# Autodesk Inventor assembly: rail_mirrored
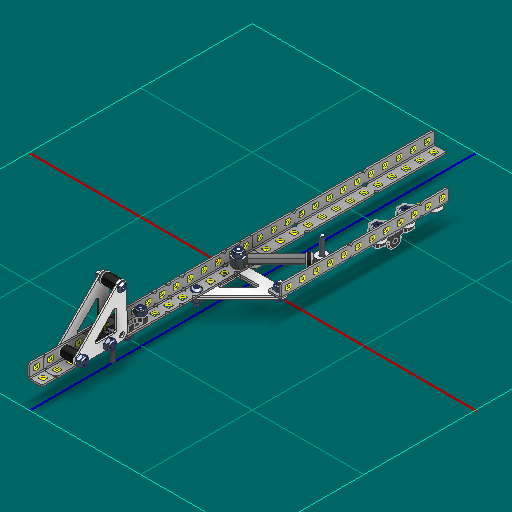
[picture p0: Inventor's stored thumbnail of the model, 512x512]
Saved by Autodesk Inventor 2025 (Build 290162000, 162)
## iProperties
Created: 2024-08-18
Part Number: rail_mirrored
Document SubType Name: Assembly
Designer: averey
Author: averey
## Documents named in this file (21)
- C:\Users\avere\vex_robotics_high_stakes\hardware\cad\ATLAS\chassis\structure\rail_mirrored\rail_mirrored.iam
- C:\Users\avere\vex_robotics_high_stakes\hardware\cad\ATLAS\chassis\structure\rail_mirrored\right_angle_gusset_mirrored.ipt
- C:\Users\avere\vex_robotics_high_stakes\hardware\cad\VEX-CAD-Inventor\Structure\Hardware\Screw Shoulder Robosource\SScrew Shoulder Smooth .500 x .18.ipt
- C:\Users\avere\vex_robotics_high_stakes\hardware\cad\VEX-CAD-Inventor\Structure\Hardware\Screw Shoulder Robosource.ipt
- C:\Users\avere\vex_robotics_high_stakes\hardware\cad\ATLAS\chassis\structure\rail_mirrored\Nut Thin Nylock_mirrored.ipt
- C:\Users\avere\vex_robotics_high_stakes\hardware\cad\ATLAS\chassis\structure\rail_mirrored\Bearing Flat Low Profile_mirrored.ipt
- C:\Users\avere\vex_robotics_high_stakes\hardware\cad\VEX-CAD-Inventor\Structure\Hardware\Screw Steel - Star\SScrew Star Smooth 1.000.ipt
- C:\Users\avere\vex_robotics_high_stakes\hardware\cad\VEX-CAD-Inventor\Structure\Hardware\Screw Steel - Star.ipt
- C:\Users\avere\vex_robotics_high_stakes\hardware\cad\VEX-CAD-Inventor\Structure\Hardware\Screw Shoulder Robosource\SScrew Shoulder Smooth .500 x .04.ipt
- C:\Users\avere\vex_robotics_high_stakes\hardware\cad\ATLAS\chassis\structure\rail_mirrored\Alu Angle 1x1x28_mirrored.ipt
- C:\Users\avere\vex_robotics_high_stakes\hardware\cad\ATLAS\chassis\structure\rail_mirrored\Alu Angle 1x1x15_mirrored.ipt
- C:\Users\avere\vex_robotics_high_stakes\hardware\cad\VEX-CAD-Inventor\Motion\Spacers\Spacer Nylon .500 OD\NSpacer White .500 OD x .125.ipt
- C:\Users\avere\vex_robotics_high_stakes\hardware\cad\VEX-CAD-Inventor\Motion\Spacers\Spacer Nylon .500 OD.ipt
- C:\Users\avere\vex_robotics_high_stakes\hardware\cad\VEX-CAD-Inventor\Structure\Hardware\Screw Steel - Star\SScrew Star Smooth .750.ipt
- C:\Users\avere\vex_robotics_high_stakes\hardware\cad\VEX-CAD-Inventor\Structure\Angle\Aluminum 1x1\Alu Angle 1x1x16.ipt
- C:\Users\avere\vex_robotics_high_stakes\hardware\cad\VEX-CAD-Inventor\Structure\Angle\Aluminum 1x1\Alu Angle 1x1x12.ipt
- C:\Users\avere\vex_robotics_high_stakes\hardware\cad\ATLAS\chassis\structure\standoff_brace_triangle.iam
- C:\Users\avere\vex_robotics_high_stakes\hardware\cad\VEX-CAD-Inventor\Motion\Shaft LS\LS Pillow Bearing Block.ipt
- C:\Users\avere\vex_robotics_high_stakes\hardware\cad\_quick_assemblies\hex_nut_retainer_w_lock_nut.iam
- C:\Users\avere\vex_robotics_high_stakes\hardware\cad\ATLAS\tower\structure\triangle_brace_mirrored.iam
- C:\Users\avere\vex_robotics_high_stakes\hardware\cad\VEX-CAD-Inventor\Structure\Hardware\Nut Thin Nylock.ipt
## Components (29 placed, 17 different names)
1. right_angle_gusset_mirrored:1 — Mate:3, Mate:5, Insert:19, Insert:20
2. right_angle_gusset_mirrored:2 — Mate:3, Mate:5, Insert:11, Insert:12, Insert:23
3. SScrew Shoulder Smooth .500 x .18:1 — Insert:20
4. SScrew Shoulder Smooth .500 x .18:2 — Insert:11, Insert:2, Insert:7
5. Nut Thin Nylock_mirrored:1 — Insert:2
6. Nut Thin Nylock_mirrored:2 — Insert:24
7. Bearing Flat Low Profile_mirrored:1 — Insert:5, Insert:4, Insert:6, Insert:21
8. SScrew Star Smooth 1.000:1 — Insert:21
9. SScrew Shoulder Smooth .500 x .04:3 — Insert:5
10. Nut Thin Nylock_mirrored:3 — Insert:4
11. Alu Angle 1x1x28_mirrored:1 — Insert:7, Insert:6, Mate:7
12. Alu Angle 1x1x15_mirrored:1 — Angle:2, Mate:7, Angle:1, Mate:6, Insert:12, Insert:14, Mate:8
13. SScrew Star Smooth 1.000:2
14. NSpacer White .500 OD x .125:1 — Insert:14, Insert:22
15. NSpacer White .500 OD x .125:2 — Insert:27
16. Nut Thin Nylock_mirrored:4
17. SScrew Star Smooth .750:3 — Insert:19
18. Alu Angle 1x1x16:1 — Insert:22, Mate:8, Insert:25, Insert:36, Mate:13, Insert:37
19. Alu Angle 1x1x12:1 — Insert:23, Insert:24, Mate:9, Insert:27, Insert:30, Mate:11, Insert:34, Insert:35
20. standoff_brace_triangle:1 [sub-assembly] — Insert:25, Mate:9
21. LS Pillow Bearing Block:1 — Insert:31, Insert:32
22. NSpacer White .500 OD x .125:3 — Insert:32, Mate:11, Mate:12
23. NSpacer White .500 OD x .125:4 — Insert:30, Insert:31
24. SScrew Shoulder Smooth .500 x .18:4
25. SScrew Shoulder Smooth .500 x .18:5
26. hex_nut_retainer_w_lock_nut:1 [sub-assembly] — Insert:34
27. hex_nut_retainer_w_lock_nut:2 [sub-assembly] — Mate:12, Insert:35
28. triangle_brace_mirrored:1 [sub-assembly] — Insert:36, Mate:13
29. Nut Thin Nylock:1 — Insert:37
## Relationships (37: Insert 25, Mate 10, Angle 2)
- Mate:3: right_angle_gusset_mirrored:1 ↔ right_angle_gusset_mirrored:2
- Mate:5: right_angle_gusset_mirrored:1 ↔ right_angle_gusset_mirrored:2
- Insert:11 (1.5875 mm): right_angle_gusset_mirrored:2 ↔ SScrew Shoulder Smooth .500 x .18:2
- Insert:2: SScrew Shoulder Smooth .500 x .18:2 ↔ Nut Thin Nylock_mirrored:1
- Insert:5 (1.5875 mm): Bearing Flat Low Profile_mirrored:1 ↔ SScrew Shoulder Smooth .500 x .04:3
- Insert:4 (1.27 mm): Bearing Flat Low Profile_mirrored:1 ↔ Nut Thin Nylock_mirrored:3
- Insert:7: SScrew Shoulder Smooth .500 x .18:2 ↔ Alu Angle 1x1x28_mirrored:1
- Insert:6: Bearing Flat Low Profile_mirrored:1 ↔ Alu Angle 1x1x28_mirrored:1
- Angle:2 (0 deg): Alu Angle 1x1x15_mirrored:1
- Mate:7: Alu Angle 1x1x28_mirrored:1 ↔ Alu Angle 1x1x15_mirrored:1
- Angle:1 (0 deg): Alu Angle 1x1x15_mirrored:1
- Mate:6: Alu Angle 1x1x15_mirrored:1
- Insert:12: right_angle_gusset_mirrored:2 ↔ Alu Angle 1x1x15_mirrored:1
- Insert:14: Alu Angle 1x1x15_mirrored:1 ↔ NSpacer White .500 OD x .125:1
- Insert:19 (1.5875 mm): right_angle_gusset_mirrored:1 ↔ SScrew Star Smooth .750:3
- Insert:20 (1.5875 mm): right_angle_gusset_mirrored:1 ↔ SScrew Shoulder Smooth .500 x .18:1
- Insert:21 (1.27 mm): Bearing Flat Low Profile_mirrored:1 ↔ SScrew Star Smooth 1.000:1
- Insert:22: NSpacer White .500 OD x .125:1 ↔ Alu Angle 1x1x16:1
- Mate:8: Alu Angle 1x1x15_mirrored:1 ↔ Alu Angle 1x1x16:1
- Insert:23: right_angle_gusset_mirrored:2 ↔ Alu Angle 1x1x12:1
- Insert:24: Nut Thin Nylock_mirrored:2 ↔ Alu Angle 1x1x12:1
- Insert:25: Alu Angle 1x1x16:1 ↔ standoff_brace_triangle:1
- Mate:9: Alu Angle 1x1x12:1 ↔ standoff_brace_triangle:1
- Insert:27: NSpacer White .500 OD x .125:2 ↔ Alu Angle 1x1x12:1
- [Insert]: LS Pillow Bearing Block:1 ↔ SScrew Shoulder Smooth .500 x .18:4
- [Insert]: LS Pillow Bearing Block:1 ↔ SScrew Shoulder Smooth .500 x .18:5
- [Mate]: NSpacer White .500 OD x .125:4 ↔ hex_nut_retainer_w_lock_nut:1
- Insert:30: Alu Angle 1x1x12:1 ↔ NSpacer White .500 OD x .125:4
- Insert:31: LS Pillow Bearing Block:1 ↔ NSpacer White .500 OD x .125:4
- Insert:32: LS Pillow Bearing Block:1 ↔ NSpacer White .500 OD x .125:3
- Mate:11: Alu Angle 1x1x12:1 ↔ NSpacer White .500 OD x .125:3
- Mate:12: NSpacer White .500 OD x .125:3 ↔ hex_nut_retainer_w_lock_nut:2
- Insert:34: Alu Angle 1x1x12:1 ↔ hex_nut_retainer_w_lock_nut:1
- Insert:35: Alu Angle 1x1x12:1 ↔ hex_nut_retainer_w_lock_nut:2
- Insert:36: Alu Angle 1x1x16:1 ↔ triangle_brace_mirrored:1
- Mate:13: Alu Angle 1x1x16:1 ↔ triangle_brace_mirrored:1
- Insert:37: Alu Angle 1x1x16:1 ↔ Nut Thin Nylock:1
